# Autodesk Inventor assembly: RCT-T001
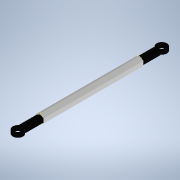
[picture p0: Inventor's stored thumbnail of the model, 180x180]
Saved by Autodesk Inventor 2020 (Build 240168000, 168)
## iProperties
Created: 2019-12-06
Part Number: RCT-T001
Document SubType Name: Assembly
Designer: Frederich Schnëider
Author: Frederich Schnëider
## Documents named in this file (3)
- C:\Users\Frederich Schnëider\Documents\GitHub\autobot\robot_model\RCT-T001.iam
- C:\Users\Frederich Schnëider\Documents\GitHub\autobot\robot_model\RCT-T001.ipt
- C:\Users\Frederich Schnëider\Documents\GitHub\autobot\robot_model\RCT-T003 (2).ipt
## Components (3 placed, 2 different names)
1. RCT-T001:1 — Coincidencia:1, Nivelación:1, Nivelación:2, Coincidencia:2, Nivelación:3, Nivelación:4
2. RCT-T003 (2):1 — Coincidencia:2, Nivelación:3, Nivelación:4
3. RCT-T003 (2):2 — Coincidencia:1, Nivelación:1, Nivelación:2
## Relationships (6: Flush 4, Mate 2)
- Coincidencia:1 [Mate]: RCT-T001:1 ↔ RCT-T003 (2):2
- Nivelación:1 [Flush] (0.4545 mm): RCT-T001:1 ↔ RCT-T003 (2):2
- Nivelación:2 [Flush] (-0.455 mm): RCT-T001:1 ↔ RCT-T003 (2):2
- Coincidencia:2 [Mate]: RCT-T001:1 ↔ RCT-T003 (2):1
- Nivelación:3 [Flush] (-0.455 mm): RCT-T001:1 ↔ RCT-T003 (2):1
- Nivelación:4 [Flush] (-0.455 mm): RCT-T001:1 ↔ RCT-T003 (2):1
